# Autodesk Inventor assembly: Gripper_Assembly
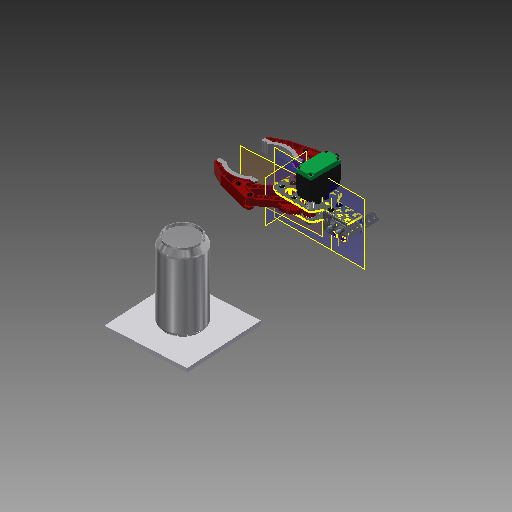
[picture p0: Inventor's stored thumbnail of the model, 512x512]
Saved by Autodesk Inventor 2018 (Build 220112000, 112)
## iProperties
Created: 2007-10-23
Part Number: Gripper_Assembly
Document SubType Name: Assembly
Designer: Tyler
Author: Tyler
## Documents named in this file (18)
- C:\Users\USER\Downloads\Inventor_2013_VEX_ KOP_-_Metric\Metric\Motion\Claw Kit.iam
- C:\Users\USER\Downloads\Inventor_2013_VEX_ KOP_-_Metric\Metric\Motion\Components\VEX-12-TOOTH-GEAR.ipt
- C:\Users\USER\Downloads\Inventor_2013_VEX_ KOP_-_Metric\Metric\Motion\Components\Vexplorer-CLAW-GEAR-LINKAGE.ipt
- C:\Users\USER\Downloads\Inventor_2013_VEX_ KOP_-_Metric\Metric\Motion\Components\Vexplorer-CLAW-LINKAGE.ipt
- C:\Users\USER\Downloads\Inventor_2013_VEX_ KOP_-_Metric\Metric\Motion\Components\SHAFT-2000.ipt
- C:\Users\USER\Downloads\Inventor_2013_VEX_ KOP_-_Metric\Metric\Motion\Components\Gripper_Assembly_SubAssembly.iam
- C:\Users\USER\Downloads\Inventor_2013_VEX_ KOP_-_Metric\Metric\Motion\Base_01.ipt
- C:\Users\USER\Downloads\Inventor_2013_VEX_ KOP_-_Metric\Metric\Motion\Can.ipt
- C:\Users\USER\Downloads\Inventor_2013_VEX_ KOP_-_Metric\Metric\Motion\Components\VEX Claw Finger.iam
- C:\Users\USER\Downloads\Inventor_2013_VEX_ KOP_-_Metric\Metric\Motion\Components\CLAW-PIN.ipt
- C:\Users\USER\Downloads\Inventor_2013_VEX_ KOP_-_Metric\Metric\Motion\Components\CLAW-SNAP.ipt
- C:\Users\USER\Downloads\Inventor_2013_VEX_ KOP_-_Metric\Metric\Motion\Components\CLAW-PIN-LONG.ipt
- C:\Users\USER\Downloads\Inventor_2013_VEX_ KOP_-_Metric\Metric\Motion\Components\VL-GUSSET-45 RevA.ipt
- C:\Users\USER\Downloads\Inventor_2013_VEX_ KOP_-_Metric\Metric\Motion\Components\SCREW-832-1500.ipt
- C:\Users\USER\Downloads\Inventor_2013_VEX_ KOP_-_Metric\Metric\Motion\Components\NUT-832-NYLOCK.ipt
- C:\Users\USER\Downloads\Inventor_2013_VEX_ KOP_-_Metric\Metric\Motion\Shaft Collar.iam
- C:\Users\USER\Downloads\Inventor_2013_VEX_ KOP_-_Metric\Metric\Motion\2 Wire Motor 393.iam
- C:\Users\USER\Downloads\Inventor_2013_VEX_ KOP_-_Metric\Metric\Motion\Components\SCREW-832_SBS0832-0250ZB.ipt
## Components (37 placed, 17 different names)
1. VEX-12-TOOTH-GEAR — Mate:62, Rotation:1, Angle:3, Flush:17, Insert:34
2. Vexplorer-CLAW-GEAR-LINKAGE — Flush:14, Rotation:2, Mate:117, Insert:9, Flush:17
3. Vexplorer-CLAW-LINKAGE — Flush:13, Angle:1, Mate:114, Insert:6, Insert:30, Mate:122
4. Vexplorer-CLAW-LINKAGE — Flush:14, Angle:2, Mate:116, Mate:118, Insert:8
5. Vexplorer-CLAW-GEAR-LINKAGE — Flush:13, Rotation:1, Rotation:2, Angle:3, Mate:113, Insert:7
6. SHAFT-2000 — Mate:62, Flush:4, Mate:123
7. Gripper_Assembly_SubAssembly:1 [sub-assembly] — Flush:4, Drive Me 1, Mate:90, Angle:1, Angle:2, Mate:113, Mate:114, Mate:116, Mate:117, Mate:118, Mate:120, Angle:6, Insert:31, Insert:32, Insert:33, Mate:122, Mate:123, Insert:34, Insert:35, Insert:36, Mate:126, Insert:39, Insert:41, Angle:7, Mate:127, Mate:129, Mate:131, Mate:133
8. Base_01:1 — Drive Me 3, Mate:89, Drive Me 1, Mate:90
9. Can:1 — Drive Me 3, Mate:89
10. VEX Claw Finger:1 [sub-assembly] — Insert:6, Insert:7, Mate:121, Insert:28, Insert:29
11. VEX Claw Finger:2 [sub-assembly] — Insert:8, Insert:9, Flush:16, Insert:26, Insert:27
12. CLAW-SNAP:1 — Insert:14
13. CLAW-SNAP:2 — Insert:15
14. CLAW-SNAP:3 — Insert:16
15. CLAW-SNAP:4 — Insert:17
16. CLAW-SNAP:5 — Insert:22
17. CLAW-SNAP:6 — Insert:23
18. CLAW-SNAP:7 — Insert:24
19. CLAW-SNAP:8 — Insert:25
20. CLAW-PIN-LONG:1 — Insert:16, Insert:26
21. CLAW-PIN-LONG:2 — Insert:17, Insert:27
22. CLAW-PIN-LONG:3 — Insert:14, Insert:28
23. CLAW-PIN-LONG:4 — Insert:15, Insert:29
24. CLAW-PIN:1 — Insert:24, Insert:31
25. CLAW-PIN:2 — Insert:25, Insert:32
26. CLAW-PIN:3 — Insert:22, Insert:30
27. CLAW-PIN:4 — Insert:23, Insert:33
28. VL-GUSSET-45 RevA:1 — Mate:124, Mate:125, Mate:126, Insert:37, Insert:38
29. VL-GUSSET-45 RevA:2 — Insert:35, Insert:36, Mate:124, Mate:125, Insert:40
30. SCREW-832-1500:1 — Insert:37
31. SCREW-832-1500:2 — Insert:38
32. NUT-832-NYLOCK:1 — Insert:40
33. NUT-832-NYLOCK:2 — Insert:39
34. Shaft Collar:1 [sub-assembly] — Insert:41, Angle:7, Mate:128
35. 2 Wire Motor 393:1 [sub-assembly] — Mate:127, Mate:128, Mate:129, Mate:134, Mate:135
36. SCREW-832_SBS0832-0250ZB:1 — Mate:131, Mate:134
37. SCREW-832_SBS0832-0250ZB:2 — Mate:133, Mate:135
## Relationships (64: Insert 28, Mate 23, Flush 6, Angle 5, RelateRotation 2)
- Drive Me 1 [Flush] (152.4 mm): Gripper_Assembly_SubAssembly:1 ↔ Base_01:1
- Mate:62: VEX-12-TOOTH-GEAR ↔ SHAFT-2000
- Flush:4 (-8.255 mm): SHAFT-2000 ↔ Gripper_Assembly_SubAssembly:1
- Drive Me 3 [Mate]: Base_01:1 ↔ Can:1
- Mate:89: Base_01:1 ↔ Can:1
- Flush:13: Vexplorer-CLAW-LINKAGE ↔ Vexplorer-CLAW-GEAR-LINKAGE
- Flush:14: Vexplorer-CLAW-GEAR-LINKAGE ↔ Vexplorer-CLAW-LINKAGE
- Mate:90: Gripper_Assembly_SubAssembly:1 ↔ Base_01:1
- Angle:1 (15 deg): Vexplorer-CLAW-LINKAGE ↔ Gripper_Assembly_SubAssembly:1
- Angle:2 (15 deg): Vexplorer-CLAW-LINKAGE ↔ Gripper_Assembly_SubAssembly:1
- Rotation:1 [RelateRotation] (0.3 ul): VEX-12-TOOTH-GEAR ↔ Vexplorer-CLAW-GEAR-LINKAGE
- Rotation:2 [RelateRotation] (1 ul): Vexplorer-CLAW-GEAR-LINKAGE
- Angle:3 (0 deg): VEX-12-TOOTH-GEAR ↔ Vexplorer-CLAW-GEAR-LINKAGE
- Mate:113: Vexplorer-CLAW-GEAR-LINKAGE ↔ Gripper_Assembly_SubAssembly:1
- Mate:114: Vexplorer-CLAW-LINKAGE ↔ Gripper_Assembly_SubAssembly:1
- Mate:116: Vexplorer-CLAW-LINKAGE ↔ Gripper_Assembly_SubAssembly:1
- Mate:117: Vexplorer-CLAW-GEAR-LINKAGE ↔ Gripper_Assembly_SubAssembly:1
- Mate:118: Vexplorer-CLAW-LINKAGE ↔ Gripper_Assembly_SubAssembly:1
- Insert:6: Vexplorer-CLAW-LINKAGE ↔ VEX Claw Finger:1
- Insert:7: Vexplorer-CLAW-GEAR-LINKAGE ↔ VEX Claw Finger:1
- Insert:8: Vexplorer-CLAW-LINKAGE ↔ VEX Claw Finger:2
- Insert:9: Vexplorer-CLAW-GEAR-LINKAGE ↔ VEX Claw Finger:2
- Mate:120: Gripper_Assembly_SubAssembly:1
- Angle:6 (0 deg): Gripper_Assembly_SubAssembly:1
- Mate:121: VEX Claw Finger:1
- Flush:16: VEX Claw Finger:2
- Insert:14: CLAW-SNAP:1 ↔ CLAW-PIN-LONG:3
- Insert:15: CLAW-SNAP:2 ↔ CLAW-PIN-LONG:4
- Insert:16: CLAW-SNAP:3 ↔ CLAW-PIN-LONG:1
- Insert:17: CLAW-SNAP:4 ↔ CLAW-PIN-LONG:2
- Insert:22: CLAW-SNAP:5 ↔ CLAW-PIN:3
- Insert:23: CLAW-SNAP:6 ↔ CLAW-PIN:4
- Insert:24: CLAW-SNAP:7 ↔ CLAW-PIN:1
- Insert:25: CLAW-SNAP:8 ↔ CLAW-PIN:2
- Insert:26: VEX Claw Finger:2 ↔ CLAW-PIN-LONG:1
- Insert:27: VEX Claw Finger:2 ↔ CLAW-PIN-LONG:2
- Insert:28: VEX Claw Finger:1 ↔ CLAW-PIN-LONG:3
- Insert:29: VEX Claw Finger:1 ↔ CLAW-PIN-LONG:4
- Insert:30: Vexplorer-CLAW-LINKAGE ↔ CLAW-PIN:3
- Insert:31: Gripper_Assembly_SubAssembly:1 ↔ CLAW-PIN:1
- Insert:32: Gripper_Assembly_SubAssembly:1 ↔ CLAW-PIN:2
- Insert:33: Gripper_Assembly_SubAssembly:1 ↔ CLAW-PIN:4
- Mate:122: Vexplorer-CLAW-LINKAGE ↔ Gripper_Assembly_SubAssembly:1
- Mate:123: SHAFT-2000 ↔ Gripper_Assembly_SubAssembly:1
- Flush:17: VEX-12-TOOTH-GEAR ↔ Vexplorer-CLAW-GEAR-LINKAGE
- Insert:34: VEX-12-TOOTH-GEAR ↔ Gripper_Assembly_SubAssembly:1
- Insert:35: Gripper_Assembly_SubAssembly:1 ↔ VL-GUSSET-45 RevA:2
- Insert:36: Gripper_Assembly_SubAssembly:1 ↔ VL-GUSSET-45 RevA:2
- Mate:124: VL-GUSSET-45 RevA:1 ↔ VL-GUSSET-45 RevA:2
- Mate:125: VL-GUSSET-45 RevA:1 ↔ VL-GUSSET-45 RevA:2
- Mate:126: Gripper_Assembly_SubAssembly:1 ↔ VL-GUSSET-45 RevA:1
- Insert:37: VL-GUSSET-45 RevA:1 ↔ SCREW-832-1500:1
- Insert:38: VL-GUSSET-45 RevA:1 ↔ SCREW-832-1500:2
- Insert:39: Gripper_Assembly_SubAssembly:1 ↔ NUT-832-NYLOCK:2
- Insert:40: VL-GUSSET-45 RevA:2 ↔ NUT-832-NYLOCK:1
- Insert:41: Gripper_Assembly_SubAssembly:1 ↔ Shaft Collar:1
- Angle:7 (180 deg): Gripper_Assembly_SubAssembly:1 ↔ Shaft Collar:1
- Mate:127: Gripper_Assembly_SubAssembly:1 ↔ 2 Wire Motor 393:1
- Mate:128: Shaft Collar:1 ↔ 2 Wire Motor 393:1
- Mate:129: Gripper_Assembly_SubAssembly:1 ↔ 2 Wire Motor 393:1
- Mate:131: Gripper_Assembly_SubAssembly:1 ↔ SCREW-832_SBS0832-0250ZB:1
- Mate:133: Gripper_Assembly_SubAssembly:1 ↔ SCREW-832_SBS0832-0250ZB:2
- Mate:134: 2 Wire Motor 393:1 ↔ SCREW-832_SBS0832-0250ZB:1
- Mate:135: 2 Wire Motor 393:1 ↔ SCREW-832_SBS0832-0250ZB:2
## Named parameters: angle = 15 deg
